# Autodesk Inventor assembly: Machine_Setup_Facing
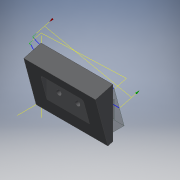
[picture p0: Inventor's stored thumbnail of the model, 180x180]
Saved by Autodesk Inventor 2018.3 (Build 223284000, 284)
## iProperties
Created: 2018-12-11
Part Number: Machine_Setup_Facing
Project: =<Part Number>
Document SubType Name: Assembly
Designer: machinetools
Author: machinetools
## Documents named in this file (3)
- R:\CAD\~Aquafil~\7407 - 456 Slant Blades-72 Flat Blades (Standard Size)\CAD\Machine_Setup_Facing.iam
- R:\CAD\~Aquafil~\7407 - 456 Slant Blades-72 Flat Blades (Standard Size)\CAD\Vice Fixture.ipt
- R:\CAD\~Aquafil~\7407 - 456 Slant Blades-72 Flat Blades (Standard Size)\CAD\DHC-1500-FF-02-003.ipt
## Components (2 placed, 2 different names)
1. Vice Fixture:1 — Mate:1, Mate:2, Mate:3
2. DHC-1500-FF-02-003:1 — Mate:1, Mate:2, Mate:3
## Relationships (3: Mate 3)
- Mate:1: Vice Fixture:1 ↔ DHC-1500-FF-02-003:1
- Mate:2: Vice Fixture:1 ↔ DHC-1500-FF-02-003:1
- Mate:3: Vice Fixture:1 ↔ DHC-1500-FF-02-003:1
